# Autodesk Inventor assembly: Chestbox_with_electronical_devices
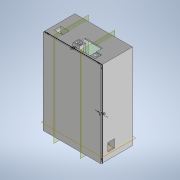
[picture p0: Inventor's stored thumbnail of the model, 180x180]
Saved by Autodesk Inventor 2021 (Build 250183000, 183)
## iProperties
Created: 2021-12-04
Part Number: Chestbox_with_electronical_devices
Document SubType Name: Assembly
Designer: marcin
Author: marcin
## Documents named in this file (4)
- C:\Users\marcin\Desktop\Motion_capture\MAIN\Models_3D\Chest_box\Chestbox_with_electronical_devices.iam
- C:\Users\marcin\Desktop\Motion_capture\MAIN\Models_3D\Chest_box\chestbox.ipt
- C:\Users\marcin\Desktop\Motion_capture\MAIN\Models_3D\Chest_box\ArduinoMega_STEP_AP203.ipt
- C:\Users\marcin\Desktop\Motion_capture\MAIN\Models_3D\Chest_box\TCA9548A Adfruit with Header.iam
## Components (3 placed, 3 different names)
1. chestbox:1 — Mate:1, Flush:1, Mate:2, Mate:3, Mate:4, Mate:5, Mate:6, Mate:7, Mate:8
2. ArduinoMega_STEP_AP203:1 — Mate:3, Mate:4, Mate:5
3. TCA9548A Adfruit with Header:1 [sub-assembly] — Mate:6, Mate:7, Mate:8
## Relationships (9: Mate 8, Flush 1)
- Mate:1: chestbox:1
- Flush:1: chestbox:1
- Mate:2: chestbox:1
- Mate:3: chestbox:1 ↔ ArduinoMega_STEP_AP203:1
- Mate:4: chestbox:1 ↔ ArduinoMega_STEP_AP203:1
- Mate:5 (10 mm): chestbox:1 ↔ ArduinoMega_STEP_AP203:1
- Mate:6 (30 mm): chestbox:1 ↔ TCA9548A Adfruit with Header:1
- Mate:7 (20 mm): chestbox:1 ↔ TCA9548A Adfruit with Header:1
- Mate:8: chestbox:1 ↔ TCA9548A Adfruit with Header:1
